# Autodesk Inventor assembly: Shooter_Assembly
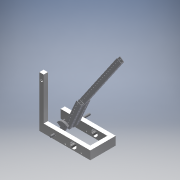
[picture p0: Inventor's stored thumbnail of the model, 180x180]
Saved by Autodesk Inventor 2019 (Build 230136000, 136)
## iProperties
Created: 2019-04-04
Part Number: Shooter_Assembly
Document SubType Name: Assembly
Designer: Delta
Author: Delta
## Documents named in this file (10)
- C:\Robotics\2019-20_CAD\offseason\random ideas\Shooter_Assembly.iam
- C:\Robotics\2019-20_CAD\offseason\random ideas\shooter.ipt
- shooter base.ipt
- C:\Robotics\2019-20_CAD\offseason\random ideas\Shooter_Stop.ipt
- C:\Robotics\COTSParts\Actobotics\585 parts\585384.ipt
- C:\Robotics\2019-20_CAD\offseason\random ideas\Shooter_Stop_Clearence.ipt
- C:\Robotics\COTSParts\Actobotics\634 parts\634064.ipt
- C:\Robotics\COTSParts\Actobotics\634 parts\634068.25inDShaft2inLong.ipt
- C:\Robotics\2019-20_CAD\offseason\random ideas\Stop.ipt
- C:\Robotics\COTSParts\Actobotics\585 parts\585396MiniChannel7.7in.ipt
## Components (10 placed, 8 different names)
1. Shooter_Stop:1 — Insert:2, Insert:4, Insert:6
2. 585384:1 — Insert:6, Insert:8
3. shooter base:1 — Mate:1, Mate:2
4. Shooter_Stop_Clearence:1 — Insert:1, Insert:3, Insert:5
5. 634064:1 — Mate:2, Insert:2
6. 634068.25inDShaft2inLong:1 — Mate:1, Insert:1
7. Stop:1 — Insert:3, Mate:3
8. 585384:2 — Insert:5, Insert:7
9. 585396MiniChannel7.7in:1 — Insert:7, Insert:8
10. Stop:2 — Insert:4, Mate:3
## Relationships (11: Insert 8, Mate 3)
- Mate:1: shooter base:1 ↔ 634068.25inDShaft2inLong:1
- Mate:2: shooter base:1 ↔ 634064:1
- Insert:1: Shooter_Stop_Clearence:1 ↔ 634068.25inDShaft2inLong:1
- Insert:2: Shooter_Stop:1 ↔ 634064:1
- Insert:3: Shooter_Stop_Clearence:1 ↔ Stop:1
- Insert:4: Shooter_Stop:1 ↔ Stop:2
- Insert:5 (0.127 mm): Shooter_Stop_Clearence:1 ↔ 585384:2
- Insert:6 (0.127 mm): Shooter_Stop:1 ↔ 585384:1
- Insert:7 (0.127 mm): 585384:2 ↔ 585396MiniChannel7.7in:1
- Insert:8 (0.127 mm): 585384:1 ↔ 585396MiniChannel7.7in:1
- Mate:3: Stop:1 ↔ Stop:2
